# Autodesk Inventor assembly: NASA-20
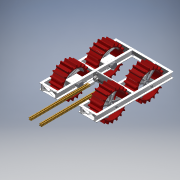
[picture p0: Inventor's stored thumbnail of the model, 180x180]
Saved by Autodesk Inventor 2020 (Build 240168000, 168)
## iProperties
RuleStatus: InUse
Created: 2019-09-05
Part Number: NASA-20
Document SubType Name: Assembly
Designer: Rick Szalay
Author: Rick Szalay
## Documents named in this file (8)
- C:\Users\Matt\OneDrive\Inventor\NASA 2020\NASA 20\NASA-20\NASA-20\NASA-20.iam
- C:\Users\Matt\OneDrive\Inventor\NASA 2020\NASA 20\NASA-20\NASA-20\FR\NASA-20-FR.iam
- C:\Users\Matt\OneDrive\Inventor\NASA 2020\NASA 20\NASA-20\NASA-20\HUB\NASA-20-HUB.iam
- C:\Users\Matt\OneDrive\Inventor\NASA 2020\NASA 20\NASA-20\NASA-20\MM\NASA-20-MM.iam
- C:\Users\Matt\OneDrive\Inventor\NASA 2020\NASA 20\NASA-20\NASA-20\5912K770_OIL-EMBEDDED MOUNTED SLEEVE BEARING.ipt
- C:\Users\Matt\OneDrive\Inventor\NASA 2020\NASA 20\NASA-20\NASA-20\2011N111_OIL-EMBEDDED THRUST BEARING.ipt
- C:\Users\Matt\OneDrive\Inventor\NASA 2020\NASA 20\NASA-20\NASA-20\9506T300_ONE-PIECE CLAMP-ON SHAFT COLLAR.ipt
- C:\Users\Matt\OneDrive\Inventor\NASA 2020\NASA 20\NASA-20\NASA-20\Bucket Assm.iam
## Components (22 placed, 7 different names)
1. NASA-20-FR:1 [sub-assembly] — Mate:20, Mate:21, Flush:13, Mate:86, Mate:87, Flush:30, Flush:31, Mate:91, Mate:92, Flush:32, Flush:33, Mate:108, Mate:109, Mate:112, Mate:113, Mate:124, Mate:125, Flush:34
2. NASA-20-HUB:1 [sub-assembly] — Flush:28, Mate:110, Mate:118
3. NASA-20-HUB:2 [sub-assembly] — Flush:28, Mate:90, Mate:111, Mate:119
4. NASA-20-HUB:3 [sub-assembly] — Flush:29, Mate:115, Mate:122
5. NASA-20-HUB:4 [sub-assembly] — Flush:29, Mate:95, Mate:114, Mate:123
6. NASA-20-MM:1 [sub-assembly] — Mate:86, Flush:31, Mate:90
7. NASA-20-MM:2 [sub-assembly] — Mate:87, Flush:30
8. NASA-20-MM:3 [sub-assembly] — Mate:92, Flush:32
9. NASA-20-MM:4 [sub-assembly] — Mate:91, Flush:33, Mate:95
10. 5912K770_OIL-EMBEDDED MOUNTED SLEEVE BEARING:1
11. 5912K770_OIL-EMBEDDED MOUNTED SLEEVE BEARING:2
12. 5912K770_OIL-EMBEDDED MOUNTED SLEEVE BEARING:3
13. 5912K770_OIL-EMBEDDED MOUNTED SLEEVE BEARING:4
14. 2011N111_OIL-EMBEDDED THRUST BEARING:1 — Mate:108, Mate:111, Mate:116
15. 2011N111_OIL-EMBEDDED THRUST BEARING:2 — Mate:109, Mate:110, Mate:117
16. 2011N111_OIL-EMBEDDED THRUST BEARING:3 — Mate:113, Mate:114, Mate:120
17. 2011N111_OIL-EMBEDDED THRUST BEARING:4 — Mate:112, Mate:115, Mate:121
18. 9506T300_ONE-PIECE CLAMP-ON SHAFT COLLAR:1 — Mate:117, Mate:118
19. 9506T300_ONE-PIECE CLAMP-ON SHAFT COLLAR:2 — Mate:116, Mate:119
20. 9506T300_ONE-PIECE CLAMP-ON SHAFT COLLAR:3 — Mate:120, Mate:123
21. 9506T300_ONE-PIECE CLAMP-ON SHAFT COLLAR:4 — Mate:121, Mate:122
22. Bucket Assm:1 [sub-assembly] — Mate:124, Mate:125, Flush:34
## Relationships (54: Mate 46, Flush 8)
- Mate:20: NASA-20-FR:1
- Mate:21: NASA-20-FR:1
- Flush:13: NASA-20-FR:1
- [Mate]: NASA-20-FR:1 ↔ NASA-20-HUB:4
- [Mate]: NASA-20-FR:1 ↔ NASA-20-HUB:3
- [Mate]: NASA-20-FR:1 ↔ NASA-20-HUB:1
- [Mate]: NASA-20-FR:1 ↔ NASA-20-HUB:2
- Flush:28: NASA-20-HUB:1 ↔ NASA-20-HUB:2
- Flush:29: NASA-20-HUB:3 ↔ NASA-20-HUB:4
- Mate:86: NASA-20-FR:1 ↔ NASA-20-MM:1
- Mate:87: NASA-20-FR:1 ↔ NASA-20-MM:2
- Flush:30: NASA-20-FR:1 ↔ NASA-20-MM:2
- [Mate]: NASA-20-FR:1 ↔ NASA-20-MM:1
- [Mate]: NASA-20-FR:1 ↔ NASA-20-MM:2
- Flush:31: NASA-20-FR:1 ↔ NASA-20-MM:1
- Mate:90 (1.5875 mm): NASA-20-HUB:2 ↔ NASA-20-MM:1
- Mate:91: NASA-20-FR:1 ↔ NASA-20-MM:4
- Mate:92: NASA-20-FR:1 ↔ NASA-20-MM:3
- Flush:32: NASA-20-FR:1 ↔ NASA-20-MM:3
- Flush:33: NASA-20-FR:1 ↔ NASA-20-MM:4
- [Mate]: NASA-20-FR:1 ↔ NASA-20-MM:4
- [Mate]: NASA-20-FR:1 ↔ NASA-20-MM:3
- Mate:95 (1.5875 mm): NASA-20-HUB:4 ↔ NASA-20-MM:4
- [Mate]: NASA-20-FR:1 ↔ 5912K770_OIL-EMBEDDED MOUNTED SLEEVE BEARING:1
- [Mate]: NASA-20-FR:1 ↔ 5912K770_OIL-EMBEDDED MOUNTED SLEEVE BEARING:1
- [Mate]: NASA-20-FR:1 ↔ 5912K770_OIL-EMBEDDED MOUNTED SLEEVE BEARING:1
- [Mate]: NASA-20-FR:1 ↔ 5912K770_OIL-EMBEDDED MOUNTED SLEEVE BEARING:2
- [Mate]: NASA-20-FR:1 ↔ 5912K770_OIL-EMBEDDED MOUNTED SLEEVE BEARING:2
- [Mate]: NASA-20-FR:1 ↔ 5912K770_OIL-EMBEDDED MOUNTED SLEEVE BEARING:2
- [Mate]: NASA-20-FR:1 ↔ 5912K770_OIL-EMBEDDED MOUNTED SLEEVE BEARING:4
- [Mate]: NASA-20-FR:1 ↔ 5912K770_OIL-EMBEDDED MOUNTED SLEEVE BEARING:3
- [Mate]: NASA-20-FR:1 ↔ 5912K770_OIL-EMBEDDED MOUNTED SLEEVE BEARING:3
- [Mate]: NASA-20-FR:1 ↔ 5912K770_OIL-EMBEDDED MOUNTED SLEEVE BEARING:4
- [Mate]: NASA-20-FR:1 ↔ 5912K770_OIL-EMBEDDED MOUNTED SLEEVE BEARING:4
- [Mate]: NASA-20-FR:1 ↔ 5912K770_OIL-EMBEDDED MOUNTED SLEEVE BEARING:3
- Mate:108: NASA-20-FR:1 ↔ 2011N111_OIL-EMBEDDED THRUST BEARING:1
- Mate:109: NASA-20-FR:1 ↔ 2011N111_OIL-EMBEDDED THRUST BEARING:2
- Mate:110: NASA-20-HUB:1 ↔ 2011N111_OIL-EMBEDDED THRUST BEARING:2
- Mate:111: NASA-20-HUB:2 ↔ 2011N111_OIL-EMBEDDED THRUST BEARING:1
- Mate:112: NASA-20-FR:1 ↔ 2011N111_OIL-EMBEDDED THRUST BEARING:4
- Mate:113: NASA-20-FR:1 ↔ 2011N111_OIL-EMBEDDED THRUST BEARING:3
- Mate:114: NASA-20-HUB:4 ↔ 2011N111_OIL-EMBEDDED THRUST BEARING:3
- Mate:115: NASA-20-HUB:3 ↔ 2011N111_OIL-EMBEDDED THRUST BEARING:4
- Mate:116: 2011N111_OIL-EMBEDDED THRUST BEARING:1 ↔ 9506T300_ONE-PIECE CLAMP-ON SHAFT COLLAR:2
- Mate:117: 2011N111_OIL-EMBEDDED THRUST BEARING:2 ↔ 9506T300_ONE-PIECE CLAMP-ON SHAFT COLLAR:1
- Mate:118: NASA-20-HUB:1 ↔ 9506T300_ONE-PIECE CLAMP-ON SHAFT COLLAR:1
- Mate:119: NASA-20-HUB:2 ↔ 9506T300_ONE-PIECE CLAMP-ON SHAFT COLLAR:2
- Mate:120: 2011N111_OIL-EMBEDDED THRUST BEARING:3 ↔ 9506T300_ONE-PIECE CLAMP-ON SHAFT COLLAR:3
- Mate:121: 2011N111_OIL-EMBEDDED THRUST BEARING:4 ↔ 9506T300_ONE-PIECE CLAMP-ON SHAFT COLLAR:4
- Mate:122: NASA-20-HUB:3 ↔ 9506T300_ONE-PIECE CLAMP-ON SHAFT COLLAR:4
- Mate:123: NASA-20-HUB:4 ↔ 9506T300_ONE-PIECE CLAMP-ON SHAFT COLLAR:3
- Mate:124: NASA-20-FR:1 ↔ Bucket Assm:1
- Mate:125 (12.7 mm): NASA-20-FR:1 ↔ Bucket Assm:1
- Flush:34 (12.7 mm): NASA-20-FR:1 ↔ Bucket Assm:1
